# Autodesk Inventor assembly: 3inModuleAssembly
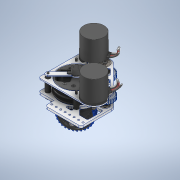
[picture p0: Inventor's stored thumbnail of the model, 180x180]
Saved by Autodesk Inventor 2020 (Build 240168000, 168)
## iProperties
Created: 2019-06-03
Part Number: 3inModuleAssembly
Document SubType Name: Assembly
Designer: Connor
Mass: 2482.46 g
Surface Area: 4233.74 cm^2
Volume: 957.958 cm^3
Density: 2.59141 g/cm^3
Author: Connor
## Documents named in this file (39)
- C:\Users\Connor\Documents\GrabCAD\2019 Robot\Swerve\TorqyoDriftV2\3inVariant\3inModuleAssembly.iam
- C:\Users\Connor\Documents\GrabCAD\2019 Robot\Swerve\TorqyoDriftV2\PlateBottom.ipt
- C:\Users\Connor\Documents\GrabCAD\2019 Robot\Swerve\TorqyoDriftV2\WheelBracketHead.ipt
- C:\Users\Connor\Documents\GrabCAD\2019 Robot\Swerve\TorqyoDriftV2\WheelBracketNut.ipt
- C:\Users\Connor\Documents\GrabCAD\2019 Robot\Swerve\TorqyoDriftV2\Imported Components\Bearings\SA035XPO.ipt
- C:\Users\Connor\Documents\GrabCAD\2019 Robot\Swerve\TorqyoDriftV2\Bevel15t.ipt
- C:\Users\Connor\Documents\GrabCAD\2019 Robot\Swerve\TorqyoDriftV2\Bevel30t.ipt
- C:\Users\Connor\Documents\GrabCAD\2019 Robot\Swerve\TorqyoDriftV2\PlanetCarriage.ipt
- C:\Users\Connor\Documents\GrabCAD\2019 Robot\Swerve\TorqyoDriftV2\RingGear.iam
- C:\Users\Connor\Documents\GrabCAD\2019 Robot\Swerve\TorqyoDriftV2\Imported Components\Spur Gears\16t_Aluminum_Spur_Gear_20_DP_3_8_Hex_Bore_217-5450.ipt
- C:\Users\Connor\Documents\GrabCAD\2019 Robot\Swerve\TorqyoDriftV2\ShortSpacer.ipt
- C:\Users\Connor\Documents\GrabCAD\2019 Robot\Swerve\TorqyoDriftV2\CarriageCap.ipt
- C:\Users\Connor\Documents\GrabCAD\2019 Robot\Swerve\TorqyoDriftV2\BearingClamp.ipt
- C:\Users\Connor\Documents\GrabCAD\2019 Robot\Swerve\TorqyoDriftV2\PlanetShaft.ipt
- C:\Users\Connor\Documents\GrabCAD\2019 Robot\Imported Components\Bearings\Radial_0.25x0.5x0.188.ipt
- C:\Users\Connor\Documents\GrabCAD\2019 Robot\Swerve\TorqyoDriftV2\TopPlate.ipt
- C:\Users\Connor\Documents\GrabCAD\2019 Robot\Swerve\TorqyoDriftV2\Imported Components\Motors\REV-21-1650.ipt
- C:\Users\Connor\Documents\GrabCAD\2019 Robot\Swerve\TorqyoDriftV2\Imported Components\Timing Pulleys\am-3263 12T 8mm Bore Pulley.ipt
- C:\Users\Connor\Documents\GrabCAD\2019 Robot\Swerve\TorqyoDriftV2\Imported Components\Sensors\TT_Electronics_Encoder_6127V1A360L.5FS.ipt
- C:\Users\Connor\Documents\GrabCAD\2019 Robot\Swerve\TorqyoDriftV2\Imported Components\Pinion Gears\12t_Steel_Spur_Gear_20_DP_CIM_Motor_217-3099.ipt
- C:\Users\Connor\Documents\GrabCAD\2019 Robot\Swerve\TorqyoDriftV2\Imported Components\Spur Gears\36t_Aluminum_Spur_Gear_20_DP_3_8_Hex_Bore_217-3213.ipt
- C:\Users\Connor\Documents\GrabCAD\2019 Robot\Swerve\TorqyoDriftV2\MotorSpacer.ipt
- C:\Users\Connor\Documents\GrabCAD\2019 Robot\Swerve\TorqyoDriftV2\DriveShaft.ipt
- C:\Users\Connor\Documents\GrabCAD\2019 Robot\Swerve\TorqyoDriftV2\Imported Components\Bolts\0.25-20_3.5in_HexHead.ipt
- C:\Users\Connor\Documents\GrabCAD\2019 Robot\Swerve\TorqyoDriftV2\Imported Components\Bolts\0.25-20_NylonLocknut.ipt
- C:\Users\Connor\Documents\GrabCAD\2019 Robot\Swerve\TorqyoDriftV2\EncoderStrip.ipt
- C:\Users\Connor\Documents\GrabCAD\2019 Robot\Swerve\TorqyoDriftV2\EncoderPinRetainer.ipt
- C:\Users\Connor\Documents\GrabCAD\2019 Robot\Swerve\TorqyoDriftV2\PlateSpacer.ipt
- C:\Users\Connor\Documents\GrabCAD\2019 Robot\Swerve\TorqyoDriftV2\EncoderStripSpacer.ipt
- C:\Users\Connor\Documents\GrabCAD\2019 Robot\Swerve\TorqyoDriftV2\PulleyShaft.ipt
- C:\Users\Connor\Documents\GrabCAD\2019 Robot\Swerve\TorqyoDriftV2\Belt.ipt
- C:\Users\Connor\Documents\GrabCAD\2019 Robot\Swerve\TorqyoDriftV2\Imported Components\Bolts\10-32_2.5in_ButtonHead.ipt
- C:\Users\Connor\Documents\GrabCAD\2019 Robot\Swerve\TorqyoDriftV2\Imported Components\Bolts\10-32_2.25in_ButtonHead.ipt
- C:\Users\Connor\Documents\GrabCAD\2019 Robot\Swerve\TorqyoDriftV2\Imported Components\Bolts\10-32_0.375in_ButtonHead.ipt
- C:\Users\Connor\Documents\GrabCAD\2019 Robot\Swerve\TorqyoDriftV2\Imported Components\Bolts\10-32_1.25in_SocketHead.ipt
- C:\Users\Connor\Documents\GrabCAD\2019 Robot\Swerve\TorqyoDriftV2\Imported Components\Bolts\10-32_1.0in_ButtonHead.ipt
- C:\Users\Connor\Documents\GrabCAD\2019 Robot\Swerve\TorqyoDriftV2\PlanetSpacer_0.5in.ipt
- C:\Users\Connor\Documents\GrabCAD\2019 Robot\Swerve\TorqyoDriftV2\Imported Components\Bearings\10_25mm_3_8_ThunderHex_ID_x_0_875_OD_x_0_280_WD_Flanged_Bearing_217-5829.ipt
- C:\Users\Connor\Documents\GrabCAD\2019 Robot\Swerve\TorqyoDriftV2\3inVariant\WheelAssembly.iam
## Components (79 placed, 38 different names)
1. PlateBottom:1 — Mate:1, Mate:2, Mate:4, Mate:7, Mate:8, Mate:38, Mate:46, Mate:47, Mate:94, Mate:96, Mate:98, Mate:100, Insert:47, Insert:48
2. WheelBracketHead:1 — Mate:2, Mate:9, Mate:14, Mate:81, Mate:82, Insert:30, Insert:32, Mate:125, Insert:53
3. WheelBracketNut:1 — Mate:4, Mate:14, Angle:1, Mate:83, Mate:84, Insert:29, Insert:31, Mate:126, Insert:51
4. SA035XPO:1 — Mate:7, Mate:8, Mate:9, Insert:1, Insert:5
5. Bevel15t:1 — Mate:20, Mate:22, Rotation:2, Mate:40, Mate:119, Mate:120, Mate:126
6. Bevel30t:1 — Mate:20, Mate:22, Flush:3, Rotation:2, Angle:8
7. Bevel15t:2 — Mate:19, Mate:21, Rotation:3, Insert:2, Angle:2, Mate:124, Mate:125
8. Bevel30t:2 — Mate:19, Mate:21, Flush:3, Rotation:3, Mate:127
9. PlanetCarriage:1 — Insert:1, Mate:31, Mate:32, Angle:1, Mate:33, Mate:35, Mate:36, Mate:39, Mate:112
10. RingGear:1 [sub-assembly] — Mate:33, Mate:34, Flush:6, Flush:8, Mate:115, Mate:116
11. RingGear:2 [sub-assembly] — Mate:31, Mate:32, Mate:34, Flush:5, Flush:7
12. 16t_Aluminum_Spur_Gear_20_DP_3_8_Hex_Bore_217-5450:1 — Mate:35, Flush:5, Angle:3, Angle:7, Insert:45
13. ShortSpacer:1 — Insert:2, Angle:2, Angle:3, Mate:43, Mate:124
14. CarriageCap:1 — Mate:36, Mate:39, Mate:69, Mate:70, Mate:93, Mate:112, Insert:40, Insert:41, Insert:42, Insert:43
15. BearingClamp:1 — Insert:5, Mate:38, Insert:23, Insert:24, Insert:25, Insert:26
16. 16t_Aluminum_Spur_Gear_20_DP_3_8_Hex_Bore_217-5450:2 — Mate:40, Flush:6
17. PlanetShaft:1 — Mate:43, Angle:7, Insert:8, Insert:52
18. PlanetShaft:2 — Insert:7, Mate:118, Insert:50
19. Radial_0.25x0.5x0.188:1 — Insert:8
20. Radial_0.25x0.5x0.188:2 — Insert:7
21. TopPlate:1 — Mate:46, Mate:47, Mate:48, Mate:51, Mate:65, Mate:66, Mate:69, Mate:71, Mate:72, Mate:73, Mate:74, Insert:15, Mate:75, Mate:85, Mate:86, Mate:88, Mate:95, Mate:97, Mate:99, Mate:101, Mate:102, Mate:104, Insert:27, Insert:28, Insert:36, Insert:37, Insert:38, Insert:39, Insert:46, Insert:49
22. REV-21-1650:1 — Mate:51, Mate:63, Mate:71, Mate:78
23. REV-21-1650:2 — Mate:48, Mate:64, Mate:72, Mate:77, Mate:79
24. am-3263 12T 8mm Bore Pulley:1 — Flush:8, Mate:68, Mate:108, Mate:121
25. am-3263 12T 8mm Bore Pulley:2 — Flush:7, Mate:67, Mate:111, Mate:122
26. TT_Electronics_Encoder_6127V1A360L.5FS:1 — Mate:70, Mate:92, Mate:93
27. 12t_Steel_Spur_Gear_20_DP_CIM_Motor_217-3099:1 — Mate:63
28. 12t_Steel_Spur_Gear_20_DP_CIM_Motor_217-3099:2 — Mate:64, Mate:79
29. 36t_Aluminum_Spur_Gear_20_DP_3_8_Hex_Bore_217-3213:1 — Mate:65, Mate:67
30. 36t_Aluminum_Spur_Gear_20_DP_3_8_Hex_Bore_217-3213:2 — Mate:66, Mate:68
31. MotorSpacer:1 — Mate:73, Mate:74, Mate:78, Mate:117
32. MotorSpacer:2 — Insert:15, Mate:75, Mate:77
33. DriveShaft:1 — Angle:8
34. 0.25-20_3.5in_HexHead:1 — Mate:81, Mate:82
35. Radial_0.25x0.5x0.188:3 — Insert:52, Insert:53
36. Radial_0.25x0.5x0.188:4 — Mate:118, Insert:50, Insert:51
37. 0.25-20_NylonLocknut:1 — Mate:83, Mate:84
38. EncoderStrip:1 — Mate:85, Mate:86, Mate:88, Mate:89, Mate:90, Mate:91, Mate:103, Mate:105
39. EncoderPinRetainer:1 — Mate:89, Mate:90, Mate:91, Mate:92
40. PlateSpacer:1 — Mate:94, Mate:95
41. PlateSpacer:2 — Mate:96, Mate:97
42. PlateSpacer:3 — Mate:100, Mate:101
43. PlateSpacer:4 — Mate:98, Mate:99
44. EncoderStripSpacer:1 — Mate:102, Mate:103
45. EncoderStripSpacer:2 — Mate:104, Mate:105
46. Belt:1 — Mate:108, Mate:115
47. Belt:2 — Mate:111, Mate:116
48. 10-32_2.5in_ButtonHead:2 — Insert:24
49. 10-32_2.5in_ButtonHead:4 — Insert:23
50. 10-32_2.25in_ButtonHead:1 — Insert:25
51. 10-32_2.25in_ButtonHead:2 — Insert:26
52. 10-32_0.375in_ButtonHead:1 — Insert:28
53. 10-32_0.375in_ButtonHead:2 — Insert:27
54. 10-32_1.25in_SocketHead:1 — Insert:29
55. 10-32_1.25in_SocketHead:2 — Insert:30
56. 10-32_1.25in_SocketHead:3 — Insert:31
57. 10-32_1.25in_SocketHead:4 — Insert:32
58. 10-32_0.375in_ButtonHead:3 — Insert:36
59. 10-32_0.375in_ButtonHead:4 — Insert:37
60. 10-32_0.375in_ButtonHead:5 — Insert:38, Mate:117
61. 10-32_0.375in_ButtonHead:6 — Insert:39
62. 10-32_1.0in_ButtonHead:1 — Insert:40
63. 10-32_1.0in_ButtonHead:2 — Insert:43
64. 10-32_1.0in_ButtonHead:3 — Insert:42
65. 10-32_1.0in_ButtonHead:4 — Insert:41
66. ShortSpacer:2 — Mate:119, Mate:120, Insert:44
67. PlanetSpacer_0.5in:1 — Insert:44
68. PlanetSpacer_0.5in:2 — Insert:45
69. 10_25mm_3_8_ThunderHex_ID_x_0_875_OD_x_0_280_WD_Flanged_Bearing_217-5829:1 — Insert:46
70. 10_25mm_3_8_ThunderHex_ID_x_0_875_OD_x_0_280_WD_Flanged_Bearing_217-5829:2 — Insert:47, Flush:9
71. 10_25mm_3_8_ThunderHex_ID_x_0_875_OD_x_0_280_WD_Flanged_Bearing_217-5829:3 — Insert:48, Flush:10
72. 10_25mm_3_8_ThunderHex_ID_x_0_875_OD_x_0_280_WD_Flanged_Bearing_217-5829:4 — Insert:49
73. PulleyShaft:1 — Mate:121, Insert:56, Insert:57, Flush:10
74. PulleyShaft:2 — Mate:122, Insert:54, Insert:55, Flush:9
75. 10-32_0.375in_ButtonHead:7 — Insert:57
76. 10-32_0.375in_ButtonHead:8 — Insert:56
77. 10-32_0.375in_ButtonHead:9 — Insert:54
78. 10-32_0.375in_ButtonHead:10 — Insert:55
79. WheelAssembly:1 [sub-assembly] — Mate:127
## Relationships (132: Mate 80, Insert 38, Flush 7, Angle 5, RelateRotation 2)
- Mate:1: PlateBottom:1
- Mate:2: PlateBottom:1 ↔ WheelBracketHead:1
- Mate:4: PlateBottom:1 ↔ WheelBracketNut:1
- Mate:7: PlateBottom:1 ↔ SA035XPO:1
- Mate:8: PlateBottom:1 ↔ SA035XPO:1
- Mate:9: WheelBracketHead:1 ↔ SA035XPO:1
- Mate:14: WheelBracketHead:1 ↔ WheelBracketNut:1
- Mate:19 (-32 mm): Bevel15t:2 ↔ Bevel30t:2
- Mate:20 (-32 mm): Bevel15t:1 ↔ Bevel30t:1
- Mate:21 (-25 mm): Bevel15t:2 ↔ Bevel30t:2
- Mate:22 (-25 mm): Bevel15t:1 ↔ Bevel30t:1
- Flush:3: Bevel30t:1 ↔ Bevel30t:2
- Rotation:2 [RelateRotation] (2 ul): Bevel15t:1 ↔ Bevel30t:1
- Rotation:3 [RelateRotation] (2 ul): Bevel15t:2 ↔ Bevel30t:2
- Insert:1: SA035XPO:1 ↔ PlanetCarriage:1
- Mate:31: PlanetCarriage:1 ↔ RingGear:2
- Mate:32: PlanetCarriage:1 ↔ RingGear:2
- Angle:1 (0 deg): WheelBracketNut:1 ↔ PlanetCarriage:1
- Mate:33: PlanetCarriage:1 ↔ RingGear:1
- Mate:34: RingGear:1 ↔ RingGear:2
- Mate:35: PlanetCarriage:1 ↔ 16t_Aluminum_Spur_Gear_20_DP_3_8_Hex_Bore_217-5450:1
- Flush:5 (0.0508 mm): RingGear:2 ↔ 16t_Aluminum_Spur_Gear_20_DP_3_8_Hex_Bore_217-5450:1
- Insert:2: Bevel15t:2 ↔ ShortSpacer:1
- Angle:2 (0 deg): Bevel15t:2 ↔ ShortSpacer:1
- Angle:3 (0 deg): 16t_Aluminum_Spur_Gear_20_DP_3_8_Hex_Bore_217-5450:1 ↔ ShortSpacer:1
- Mate:36: PlanetCarriage:1 ↔ CarriageCap:1
- Insert:5: SA035XPO:1 ↔ BearingClamp:1
- Mate:38: PlateBottom:1 ↔ BearingClamp:1
- Mate:39: PlanetCarriage:1 ↔ CarriageCap:1
- Mate:40: Bevel15t:1 ↔ 16t_Aluminum_Spur_Gear_20_DP_3_8_Hex_Bore_217-5450:2
- Flush:6 (0.0508 mm): RingGear:1 ↔ 16t_Aluminum_Spur_Gear_20_DP_3_8_Hex_Bore_217-5450:2
- Mate:43: ShortSpacer:1 ↔ PlanetShaft:1
- Angle:7 (0 deg): 16t_Aluminum_Spur_Gear_20_DP_3_8_Hex_Bore_217-5450:1 ↔ PlanetShaft:1
- Insert:7: PlanetShaft:2 ↔ Radial_0.25x0.5x0.188:2
- Insert:8: PlanetShaft:1 ↔ Radial_0.25x0.5x0.188:1
- Mate:46: PlateBottom:1 ↔ TopPlate:1
- Mate:47 (31.75 mm): PlateBottom:1 ↔ TopPlate:1
- Mate:48: TopPlate:1 ↔ REV-21-1650:2
- Mate:51: TopPlate:1 ↔ REV-21-1650:1
- Flush:7 (0.5715 mm): RingGear:2 ↔ am-3263 12T 8mm Bore Pulley:2
- Flush:8 (0.5715 mm): RingGear:1 ↔ am-3263 12T 8mm Bore Pulley:1
- Mate:63: REV-21-1650:1 ↔ 12t_Steel_Spur_Gear_20_DP_CIM_Motor_217-3099:1
- Mate:64: REV-21-1650:2 ↔ 12t_Steel_Spur_Gear_20_DP_CIM_Motor_217-3099:2
- Mate:65: TopPlate:1 ↔ 36t_Aluminum_Spur_Gear_20_DP_3_8_Hex_Bore_217-3213:1
- Mate:66: TopPlate:1 ↔ 36t_Aluminum_Spur_Gear_20_DP_3_8_Hex_Bore_217-3213:2
- Mate:67: am-3263 12T 8mm Bore Pulley:2 ↔ 36t_Aluminum_Spur_Gear_20_DP_3_8_Hex_Bore_217-3213:1
- Mate:68: am-3263 12T 8mm Bore Pulley:1 ↔ 36t_Aluminum_Spur_Gear_20_DP_3_8_Hex_Bore_217-3213:2
- Mate:69: CarriageCap:1 ↔ TopPlate:1
- Mate:70: CarriageCap:1 ↔ TT_Electronics_Encoder_6127V1A360L.5FS:1
- Mate:71: TopPlate:1 ↔ REV-21-1650:1
- Mate:72: TopPlate:1 ↔ REV-21-1650:2
- Mate:73: TopPlate:1 ↔ MotorSpacer:1
- Mate:74: TopPlate:1 ↔ MotorSpacer:1
- Insert:15: TopPlate:1 ↔ MotorSpacer:2
- Mate:75: TopPlate:1 ↔ MotorSpacer:2
- Mate:77: REV-21-1650:2 ↔ MotorSpacer:2
- Mate:78: REV-21-1650:1 ↔ MotorSpacer:1
- Mate:79: REV-21-1650:2 ↔ 12t_Steel_Spur_Gear_20_DP_CIM_Motor_217-3099:2
- Mate:81: WheelBracketHead:1 ↔ 0.25-20_3.5in_HexHead:1
- Mate:82: WheelBracketHead:1 ↔ 0.25-20_3.5in_HexHead:1
- Mate:83: WheelBracketNut:1 ↔ 0.25-20_NylonLocknut:1
- Mate:84: WheelBracketNut:1 ↔ 0.25-20_NylonLocknut:1
- Mate:85: TopPlate:1 ↔ EncoderStrip:1
- Mate:86: TopPlate:1 ↔ EncoderStrip:1
- Mate:88 (6.35 mm): TopPlate:1 ↔ EncoderStrip:1
- Mate:89: EncoderStrip:1 ↔ EncoderPinRetainer:1
- Mate:90: EncoderStrip:1 ↔ EncoderPinRetainer:1
- Mate:91: EncoderStrip:1 ↔ EncoderPinRetainer:1
- Mate:92: TT_Electronics_Encoder_6127V1A360L.5FS:1 ↔ EncoderPinRetainer:1
- Mate:93: CarriageCap:1 ↔ TT_Electronics_Encoder_6127V1A360L.5FS:1
- Mate:94: PlateBottom:1 ↔ PlateSpacer:1
- Mate:95: TopPlate:1 ↔ PlateSpacer:1
- Mate:96: PlateBottom:1 ↔ PlateSpacer:2
- Mate:97: TopPlate:1 ↔ PlateSpacer:2
- Mate:98: PlateBottom:1 ↔ PlateSpacer:4
- Mate:99: TopPlate:1 ↔ PlateSpacer:4
- Mate:100: PlateBottom:1 ↔ PlateSpacer:3
- Mate:101: TopPlate:1 ↔ PlateSpacer:3
- Mate:102: TopPlate:1 ↔ EncoderStripSpacer:1
- Mate:103: EncoderStrip:1 ↔ EncoderStripSpacer:1
- Mate:104: TopPlate:1 ↔ EncoderStripSpacer:2
- Mate:105: EncoderStrip:1 ↔ EncoderStripSpacer:2
- Mate:108: am-3263 12T 8mm Bore Pulley:1 ↔ Belt:1
- Mate:111: am-3263 12T 8mm Bore Pulley:2 ↔ Belt:2
- Angle:8 (0 deg): Bevel30t:1 ↔ DriveShaft:1
- Insert:23: BearingClamp:1 ↔ 10-32_2.5in_ButtonHead:4
- Insert:24: BearingClamp:1 ↔ 10-32_2.5in_ButtonHead:2
- Insert:25: BearingClamp:1 ↔ 10-32_2.25in_ButtonHead:1
- Insert:26: BearingClamp:1 ↔ 10-32_2.25in_ButtonHead:2
- Insert:27: TopPlate:1 ↔ 10-32_0.375in_ButtonHead:2
- Insert:28: TopPlate:1 ↔ 10-32_0.375in_ButtonHead:1
- Insert:29: WheelBracketNut:1 ↔ 10-32_1.25in_SocketHead:1
- Insert:30: WheelBracketHead:1 ↔ 10-32_1.25in_SocketHead:2
- Insert:31: WheelBracketNut:1 ↔ 10-32_1.25in_SocketHead:3
- Insert:32: WheelBracketHead:1 ↔ 10-32_1.25in_SocketHead:4
- Mate:112: PlanetCarriage:1 ↔ CarriageCap:1
- Mate:115: RingGear:1 ↔ Belt:1
- Mate:116: RingGear:1 ↔ Belt:2
- Insert:36: TopPlate:1 ↔ 10-32_0.375in_ButtonHead:3
- Insert:37: TopPlate:1 ↔ 10-32_0.375in_ButtonHead:4
- Insert:38: TopPlate:1 ↔ 10-32_0.375in_ButtonHead:5
- Insert:39: TopPlate:1 ↔ 10-32_0.375in_ButtonHead:6
- Mate:117: MotorSpacer:1 ↔ 10-32_0.375in_ButtonHead:5
- Insert:40: CarriageCap:1 ↔ 10-32_1.0in_ButtonHead:1
- Insert:41: CarriageCap:1 ↔ 10-32_1.0in_ButtonHead:4
- Insert:42: CarriageCap:1 ↔ 10-32_1.0in_ButtonHead:3
- Insert:43: CarriageCap:1 ↔ 10-32_1.0in_ButtonHead:2
- Mate:118: PlanetShaft:2 ↔ Radial_0.25x0.5x0.188:4
- Mate:119: Bevel15t:1 ↔ ShortSpacer:2
- Mate:120: Bevel15t:1 ↔ ShortSpacer:2
- Insert:44: ShortSpacer:2 ↔ PlanetSpacer_0.5in:1
- Insert:45: 16t_Aluminum_Spur_Gear_20_DP_3_8_Hex_Bore_217-5450:1 ↔ PlanetSpacer_0.5in:2
- Insert:46: TopPlate:1 ↔ 10_25mm_3_8_ThunderHex_ID_x_0_875_OD_x_0_280_WD_Flanged_Bearing_217-5829:1
- Insert:47: PlateBottom:1 ↔ 10_25mm_3_8_ThunderHex_ID_x_0_875_OD_x_0_280_WD_Flanged_Bearing_217-5829:2
- Insert:48: PlateBottom:1 ↔ 10_25mm_3_8_ThunderHex_ID_x_0_875_OD_x_0_280_WD_Flanged_Bearing_217-5829:3
- Insert:49: TopPlate:1 ↔ 10_25mm_3_8_ThunderHex_ID_x_0_875_OD_x_0_280_WD_Flanged_Bearing_217-5829:4
- Mate:121: am-3263 12T 8mm Bore Pulley:1 ↔ PulleyShaft:1
- Mate:122: am-3263 12T 8mm Bore Pulley:2 ↔ PulleyShaft:2
- Mate:124: Bevel15t:2 ↔ ShortSpacer:1
- Mate:125: WheelBracketHead:1 ↔ Bevel15t:2
- Mate:126: WheelBracketNut:1 ↔ Bevel15t:1
- Insert:50: PlanetShaft:2 ↔ Radial_0.25x0.5x0.188:4
- Insert:51: WheelBracketNut:1 ↔ Radial_0.25x0.5x0.188:4
- Insert:52: PlanetShaft:1 ↔ Radial_0.25x0.5x0.188:3
- Insert:53: WheelBracketHead:1 ↔ Radial_0.25x0.5x0.188:3
- Insert:54 (0.7937 mm): PulleyShaft:2 ↔ 10-32_0.375in_ButtonHead:9
- Insert:55 (0.7937 mm): PulleyShaft:2 ↔ 10-32_0.375in_ButtonHead:10
- Insert:56 (0.7937 mm): PulleyShaft:1 ↔ 10-32_0.375in_ButtonHead:8
- Insert:57 (0.7937 mm): PulleyShaft:1 ↔ 10-32_0.375in_ButtonHead:7
- Flush:9: 10_25mm_3_8_ThunderHex_ID_x_0_875_OD_x_0_280_WD_Flanged_Bearing_217-5829:2 ↔ PulleyShaft:2
- Flush:10: 10_25mm_3_8_ThunderHex_ID_x_0_875_OD_x_0_280_WD_Flanged_Bearing_217-5829:3 ↔ PulleyShaft:1
- Mate:127: Bevel30t:2 ↔ WheelAssembly:1
